# Autodesk Inventor assembly: VerticalSlidingCart
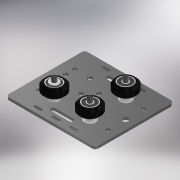
[picture p0: Inventor's stored thumbnail of the model, 180x180]
Saved by Autodesk Inventor 2020.3 (Build 243373000, 373)
## iProperties
Created: 2021-08-04
Part Number: VerticalSlidingCart
Document SubType Name: Assembly
Designer: justi
Author: justi
## Documents named in this file (6)
- F:\UQ Engineering\2021 ~ 5th Year\Semester 2\METR4911-THESIS\FarmBot CAD\FarmBotV1\VerticalSlidingCart.iam
- F:\UQ Engineering\2021 ~ 5th Year\Semester 2\METR4911-THESIS\FarmBot CAD\FarmBotV1\VSlotHardware\20mm gantry plate.ipt
- F:\UQ Engineering\2021 ~ 5th Year\Semester 2\METR4911-THESIS\FarmBot CAD\FarmBotV1\VSlotHardware\V-Wheel Kit.iam
- F:\UQ Engineering\2021 ~ 5th Year\Semester 2\METR4911-THESIS\FarmBot CAD\FarmBotV1\VSlotHardware\6mm Spacer.ipt
- F:\UQ Engineering\2021 ~ 5th Year\Semester 2\METR4911-THESIS\FarmBot CAD\FarmBotV1\VSlotHardware\Eccentric Spacer 6mm.ipt
- F:\UQ Engineering\2021 ~ 5th Year\Semester 2\METR4911-THESIS\FarmBot CAD\FarmBotV1\VSlotHardware\M5x25 low profile screw.ipt
## Components (10 placed, 5 different names)
1. 20mm gantry plate:1 — Mate:8, Mate:9, Mate:10, Mate:16, Mate:18, Mate:19, Mate:22, Mate:25, Mate:26, Mate:27
2. V-Wheel Kit:2 [sub-assembly] — Mate:11, Mate:12
3. V-Wheel Kit:3 [sub-assembly] — Mate:29
4. 6mm Spacer:2 — Mate:8, Mate:28
5. Eccentric Spacer 6mm:1 — Mate:9, Mate:10, Mate:11, Mate:12, Mate:17, Mate:25
6. V-Wheel Kit:4 [sub-assembly]
7. Eccentric Spacer 6mm:3 — Mate:16, Mate:20
8. M5x25 low profile screw:1 — Mate:19, Mate:20, Mate:26
9. M5x25 low profile screw:3 — Mate:22, Mate:27, Mate:28, Mate:29
10. M5x25 low profile screw:4 — Mate:17, Mate:18
## Relationships (19: Mate 19)
- [Mate]: V-Wheel Kit:3 ↔ 6mm Spacer:2
- Mate:8: 20mm gantry plate:1 ↔ 6mm Spacer:2
- Mate:9: 20mm gantry plate:1 ↔ Eccentric Spacer 6mm:1
- Mate:10: 20mm gantry plate:1 ↔ Eccentric Spacer 6mm:1
- Mate:11: V-Wheel Kit:2 ↔ Eccentric Spacer 6mm:1
- Mate:12: V-Wheel Kit:2 ↔ Eccentric Spacer 6mm:1
- [Mate]: V-Wheel Kit:4 ↔ Eccentric Spacer 6mm:3
- [Mate]: V-Wheel Kit:4 ↔ Eccentric Spacer 6mm:3
- Mate:16: 20mm gantry plate:1 ↔ Eccentric Spacer 6mm:3
- Mate:17: Eccentric Spacer 6mm:1 ↔ M5x25 low profile screw:4
- Mate:18: 20mm gantry plate:1 ↔ M5x25 low profile screw:4
- Mate:19: 20mm gantry plate:1 ↔ M5x25 low profile screw:1
- Mate:20: Eccentric Spacer 6mm:3 ↔ M5x25 low profile screw:1
- Mate:22: 20mm gantry plate:1 ↔ M5x25 low profile screw:3
- Mate:25: 20mm gantry plate:1 ↔ Eccentric Spacer 6mm:1
- Mate:26: 20mm gantry plate:1 ↔ M5x25 low profile screw:1
- Mate:27: 20mm gantry plate:1 ↔ M5x25 low profile screw:3
- Mate:28: 6mm Spacer:2 ↔ M5x25 low profile screw:3
- Mate:29: V-Wheel Kit:3 ↔ M5x25 low profile screw:3
## Named parameters: d4_d3 = 0 mm, d12_d10 = 0 mm, d13_d11 = 0 mm
